# Autodesk Inventor assembly: rack
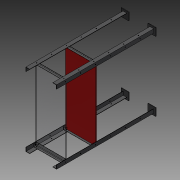
[picture p0: Inventor's stored thumbnail of the model, 180x180]
Saved by Autodesk Inventor 2018 (Build 220112000, 112)
## iProperties
Created: 2017-05-04
Part Number: rack
Document SubType Name: Assembly
Designer: AYUSH SHUKLA
Author: AYUSH SHUKLA
## Documents named in this file (4)
- C:\Study\BTP2\Robomuse Inventor CAD\Rack\rack.iam
- C:\Study\BTP2\Robomuse Inventor CAD\Rack\sides.ipt
- C:\Study\BTP2\Robomuse Inventor CAD\Rack\shelf.ipt
- C:\Study\BTP2\Robomuse Inventor CAD\Rack\pannel_small.ipt
## Components (10 placed, 3 different names)
1. sides:1
2. shelf:1
3. sides:2
4. pannel_small:1
5. sides:3
6. pannel_small:2
7. sides:4
8. shelf:2
9. pannel_small:5
10. pannel_small:6
## Relationships (23: Mate 23)
- [Mate]: shelf:1 ↔ pannel_small:1
- [Mate]: shelf:1 ↔ pannel_small:1
- [Mate]: shelf:1 ↔ pannel_small:2
- [Mate]: shelf:1 ↔ pannel_small:2
- [Mate]: shelf:1 ↔ pannel_small:2
- [Mate]: shelf:1 ↔ pannel_small:1
- [Mate]: shelf:2 ↔ pannel_small:5
- [Mate]: shelf:2 ↔ pannel_small:5
- [Mate]: shelf:2 ↔ pannel_small:6
- [Mate]: shelf:2 ↔ pannel_small:6
- [Mate]: shelf:2 ↔ pannel_small:6
- [Mate]: shelf:2 ↔ pannel_small:5
- [Mate]: sides:3 ↔ pannel_small:6
- [Mate]: sides:1 ↔ pannel_small:6
- [Mate]: sides:1 ↔ pannel_small:6
- [Mate]: sides:3 ↔ pannel_small:6
- [Mate]: sides:2 ↔ pannel_small:5
- [Mate]: sides:2 ↔ pannel_small:5
- [Mate]: sides:3 ↔ pannel_small:2
- [Mate]: sides:1 ↔ pannel_small:2
- [Mate]: sides:3 ↔ pannel_small:2
- [Mate]: sides:4 ↔ pannel_small:5
- [Mate]: sides:4 ↔ pannel_small:5
## Named parameters: d5_d11 = 0 mm, d6_d12 = 0 mm, d7_d13 = 0 mm, d8_d14 = 0 mm, d9_d15 = 0 mm, d10_d16 = 0 mm, d17_d11 = 0 mm, d18_d12 = 0 mm, d19_d13 = 0 mm, d20_d14 = 0 mm, d21_d15 = 0 mm, d22_d16 = 0 mm
